# Autodesk Inventor assembly: Frame
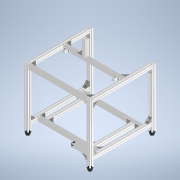
[picture p0: Inventor's stored thumbnail of the model, 180x180]
Saved by Autodesk Inventor 2020.2 (Build 242310000, 310)
## iProperties
Created: 2020-07-30
Part Number: Frame
Document SubType Name: Assembly
Designer: JK
Author: JK
## Documents named in this file (10)
- C:\Users\JK\Documents\Inventor\Anet Upgrade\Frame.iam
- C:\Users\JK\Documents\Inventor\Anet Upgrade\30x30x500.ipt
- C:\Users\JK\Documents\Inventor\Anet Upgrade\Cornerassembly.iam
- C:\Users\JK\Documents\Inventor\Anet Upgrade\SK8.iam
- C:\Users\JK\Documents\Inventor\Anet Upgrade\30x30x125.ipt
- C:\Users\JK\Documents\Inventor\Anet Upgrade\30x30x340.ipt
- C:\Users\JK\Documents\Inventor\Anet Upgrade\3030_endCap.ipt
- C:\Users\JK\Documents\Inventor\Anet Upgrade\Footassembly.iam
- C:\Users\JK\Documents\Inventor\Anet Upgrade\M5x12BoltFlatHead.ipt
- C:\Users\JK\Documents\Inventor\Anet Upgrade\T_Slot_Nut_Dropin_3030m5ipt.ipt
## Components (53 placed, 9 different names)
1. 30x30x500:9 — Flush:17, Mate:14, Flush:19, Flush:24, Mate:38, Mate:42
2. 30x30x500:10 — Flush:16, Flush:17, Mate:13, Flush:18, Mate:36, Mate:40, Flush:57
3. 30x30x500:3 — Mate:12, Flush:16, Mate:49, Flush:51, Mate:50, Flush:52, Mate:55, Mate:58, Flush:56, Flush:64, Mate:88
4. 30x30x500:4 — Mate:12, Mate:51, Mate:53
5. Cornerassembly:1 [sub-assembly]
6. Cornerassembly:2 [sub-assembly]
7. Cornerassembly:3 [sub-assembly]
8. Cornerassembly:4 [sub-assembly]
9. 30x30x500:1 — Mate:13, Flush:18, Mate:17, Flush:25, Mate:34, Mate:41, Flush:45, Mate:66, Mate:67, Flush:62, Mate:73, Angle:1, Mate:83, Flush:78
10. 30x30x500:2 — Mate:14, Flush:19, Flush:27, Mate:28, Flush:39, Flush:46, Mate:60, Mate:61, Flush:58, Flush:59, Mate:75, Angle:4, Flush:77, Mate:85, Mate:88
11. 30x30x500:5 — Flush:24, Mate:18, Mate:30, Mate:39, Flush:44, Mate:82, Flush:80
12. 30x30x500:6 — Flush:79, Flush:81, Flush:82, Mate:87, Mate:89, Flush:85, Mate:90, Mate:95
13. 30x30x500:11 — Mate:17, Flush:25, Mate:19, Mate:27, Flush:41, Flush:42, Mate:64, Flush:61, Flush:81, Flush:82, Mate:89, Mate:94, Flush:87, Mate:101
14. 30x30x500:12 — Mate:18, Flush:27, Flush:40, Flush:50, Mate:63, Flush:77, Mate:85, Flush:80, Flush:83, Mate:91, Mate:93, Angle:5, Mate:102
15. 30x30x500:7 — Mate:19, Mate:20, Flush:31, Mate:26, Flush:38, Mate:45, Flush:48, Flush:83, Flush:84, Mate:86, Flush:86, Mate:92, Flush:91
16. SK8:1 [sub-assembly] — Mate:20, Flush:31, Mate:79, Mate:80, Flush:76, Mate:84, Mate:96, Angle:5, Angle:6
17. SK8:2 [sub-assembly] — Mate:60, Mate:78, Mate:81, Flush:76, Mate:96, Flush:87, Angle:7, Angle:8
18. Cornerassembly:5 [sub-assembly] — Flush:86, Mate:92, Mate:93
19. Cornerassembly:6 [sub-assembly] — Mate:26, Mate:27, Flush:38
20. Cornerassembly:7 [sub-assembly] — Mate:28, Flush:39, Mate:102
21. Cornerassembly:8 [sub-assembly] — Mate:30, Flush:40, Mate:91
22. Cornerassembly:9 [sub-assembly] — Flush:41, Mate:94, Mate:95
23. Cornerassembly:10 [sub-assembly] — Mate:34, Flush:42, Mate:101
24. Cornerassembly:11 [sub-assembly] — Mate:36, Flush:85, Mate:90
25. Cornerassembly:13 [sub-assembly] — Mate:40, Mate:41, Flush:45
26. Cornerassembly:14 [sub-assembly] — Mate:38, Mate:39, Flush:44
27. Cornerassembly:15 [sub-assembly] — Mate:42, Flush:46
28. 30x30x125:1 — Mate:46, Flush:50, Flush:84, Mate:86
29. Cornerassembly:16 [sub-assembly] — Mate:45, Mate:46, Flush:48
30. 30x30x340:1 — Mate:49, Flush:51, Flush:54, Mate:54, Flush:55, Mate:56, Mate:59
31. 30x30x340:2 — Mate:50, Flush:52, Mate:52, Flush:53, Mate:57, Mate:59, Flush:57
32. Cornerassembly:17 [sub-assembly] — Flush:54, Mate:53, Mate:54
33. Cornerassembly:18 [sub-assembly] — Mate:57, Mate:58, Flush:56
34. Cornerassembly:19 [sub-assembly] — Mate:55, Flush:55, Mate:56
35. Cornerassembly:20 [sub-assembly] — Mate:51, Mate:52, Flush:53
36. 30x30x500:8 — Mate:61, Flush:58, Flush:59, Mate:62, Flush:60, Flush:78, Flush:79
37. Cornerassembly:21 [sub-assembly] — Mate:62, Flush:60, Mate:63
38. Cornerassembly:22 [sub-assembly] — Mate:64, Flush:61
39. Cornerassembly:23 [sub-assembly] — Mate:66, Mate:68, Flush:63, Flush:64
40. 30x30x125:2 — Mate:67, Flush:62, Mate:68, Flush:63, Mate:69, Flush:65, Flush:66
41. 3030_endCap:1 — Mate:69, Flush:65, Flush:66
42. Footassembly:1 [sub-assembly] — Mate:73, Angle:1, Flush:69, Flush:70, Flush:75, Mate:83
43. Footassembly:2 [sub-assembly] — Mate:75, Flush:69, Angle:4
44. Footassembly:3 [sub-assembly] — Flush:75, Mate:82
45. Footassembly:4 [sub-assembly] — Flush:70, Mate:87
46. M5x12BoltFlatHead:1 — Mate:78, Flush:72, Flush:73, Mate:100
47. M5x12BoltFlatHead:2 — Mate:79, Flush:74, Mate:98
48. M5x12BoltFlatHead:3 — Mate:80, Flush:73, Flush:74, Mate:84, Mate:97
49. M5x12BoltFlatHead:4 — Mate:81, Flush:72, Mate:99
50. T_Slot_Nut_Dropin_3030m5ipt:1 — Mate:97, Flush:90, Angle:6
51. T_Slot_Nut_Dropin_3030m5ipt:2 — Mate:98, Flush:89, Flush:90
52. T_Slot_Nut_Dropin_3030m5ipt:3 — Mate:99, Flush:88, Flush:89, Angle:7, Flush:91
53. T_Slot_Nut_Dropin_3030m5ipt:4 — Mate:100, Flush:88, Angle:8
## Relationships (147: Mate 78, Flush 63, Angle 6)
- [Mate]: 30x30x500:9 ↔ 30x30x500:3
- [Flush]: 30x30x500:9 ↔ 30x30x500:3
- [Mate]: 30x30x500:9 ↔ 30x30x500:4
- [Flush]: 30x30x500:9 ↔ 30x30x500:4
- [Mate]: 30x30x500:10 ↔ 30x30x500:3
- [Flush]: 30x30x500:10 ↔ 30x30x500:4
- [Mate]: 30x30x500:9 ↔ Cornerassembly:1
- [Mate]: 30x30x500:4 ↔ Cornerassembly:1
- [Flush] (0.5 mm): 30x30x500:9 ↔ Cornerassembly:1
- [Mate]: 30x30x500:3 ↔ Cornerassembly:3
- [Flush] (0.5 mm): 30x30x500:9 ↔ Cornerassembly:3
- [Mate]: 30x30x500:9 ↔ Cornerassembly:3
- [Mate]: 30x30x500:3 ↔ Cornerassembly:2
- [Mate]: 30x30x500:10 ↔ Cornerassembly:2
- [Flush] (0.5 mm): 30x30x500:10 ↔ Cornerassembly:2
- [Mate]: 30x30x500:10 ↔ Cornerassembly:4
- [Mate]: 30x30x500:4 ↔ Cornerassembly:4
- [Flush] (0.5 mm): 30x30x500:4 ↔ Cornerassembly:4
- Mate:12 (-400 mm): 30x30x500:3 ↔ 30x30x500:4
- Flush:16 (-50 mm): 30x30x500:10 ↔ 30x30x500:3
- Flush:17: 30x30x500:9 ↔ 30x30x500:10
- Mate:13: 30x30x500:10 ↔ 30x30x500:1
- Mate:14: 30x30x500:9 ↔ 30x30x500:2
- Flush:18: 30x30x500:10 ↔ 30x30x500:1
- Flush:19: 30x30x500:9 ↔ 30x30x500:2
- Flush:24: 30x30x500:9 ↔ 30x30x500:5
- Mate:17: 30x30x500:1 ↔ 30x30x500:11
- Flush:25: 30x30x500:1 ↔ 30x30x500:11
- Mate:18: 30x30x500:5 ↔ 30x30x500:12
- Flush:27: 30x30x500:2 ↔ 30x30x500:12
- Mate:19: 30x30x500:11 ↔ 30x30x500:7
- Mate:20: 30x30x500:7 ↔ SK8:1
- Flush:31 (8 mm): 30x30x500:7 ↔ SK8:1
- Mate:26: 30x30x500:7 ↔ Cornerassembly:6
- Mate:27: 30x30x500:11 ↔ Cornerassembly:6
- Flush:38 (0.5 mm): 30x30x500:7 ↔ Cornerassembly:6
- Mate:28: 30x30x500:2 ↔ Cornerassembly:7
- Flush:39 (0.5 mm): 30x30x500:2 ↔ Cornerassembly:7
- Mate:30: 30x30x500:5 ↔ Cornerassembly:8
- Flush:40 (0.5 mm): 30x30x500:12 ↔ Cornerassembly:8
- Flush:41 (0.5 mm): 30x30x500:11 ↔ Cornerassembly:9
- Mate:34: 30x30x500:1 ↔ Cornerassembly:10
- Flush:42 (0.5 mm): 30x30x500:11 ↔ Cornerassembly:10
- Mate:36: 30x30x500:10 ↔ Cornerassembly:11
- Mate:38: 30x30x500:9 ↔ Cornerassembly:14
- Mate:39: 30x30x500:5 ↔ Cornerassembly:14
- Flush:44 (0.5 mm): 30x30x500:5 ↔ Cornerassembly:14
- Mate:40: 30x30x500:10 ↔ Cornerassembly:13
- Mate:41: 30x30x500:1 ↔ Cornerassembly:13
- Flush:45 (0.5 mm): 30x30x500:1 ↔ Cornerassembly:13
- Mate:42: 30x30x500:9 ↔ Cornerassembly:15
- Flush:46 (0.5 mm): 30x30x500:2 ↔ Cornerassembly:15
- Mate:45: 30x30x500:7 ↔ Cornerassembly:16
- Mate:46: 30x30x125:1 ↔ Cornerassembly:16
- Flush:48 (0.5 mm): 30x30x500:7 ↔ Cornerassembly:16
- Flush:50 (190 mm): 30x30x500:12 ↔ 30x30x125:1
- Mate:49: 30x30x500:3 ↔ 30x30x340:1
- Flush:51: 30x30x500:3 ↔ 30x30x340:1
- Mate:50: 30x30x500:3 ↔ 30x30x340:2
- Flush:52: 30x30x500:3 ↔ 30x30x340:2
- Mate:51: 30x30x500:4 ↔ Cornerassembly:20
- Mate:52: 30x30x340:2 ↔ Cornerassembly:20
- Flush:53: 30x30x340:2 ↔ Cornerassembly:20
- Flush:54 (0.5 mm): 30x30x340:1 ↔ Cornerassembly:17
- Mate:53: 30x30x500:4 ↔ Cornerassembly:17
- Mate:54: 30x30x340:1 ↔ Cornerassembly:17
- Mate:55: 30x30x500:3 ↔ Cornerassembly:19
- Flush:55 (0.5 mm): 30x30x340:1 ↔ Cornerassembly:19
- Mate:56: 30x30x340:1 ↔ Cornerassembly:19
- Mate:57: 30x30x340:2 ↔ Cornerassembly:18
- Mate:58: 30x30x500:3 ↔ Cornerassembly:18
- Flush:56 (0.5 mm): 30x30x500:3 ↔ Cornerassembly:18
- Mate:59 (362 mm): 30x30x340:1 ↔ 30x30x340:2
- Flush:57 (69 mm): 30x30x500:10 ↔ 30x30x340:2
- Mate:60 (-280 mm): 30x30x500:2 ↔ SK8:2
- Mate:61: 30x30x500:2 ↔ 30x30x500:8
- Flush:58: 30x30x500:2 ↔ 30x30x500:8
- Flush:59: 30x30x500:2 ↔ 30x30x500:8
- Mate:62: 30x30x500:8 ↔ Cornerassembly:21
- Flush:60 (0.5 mm): 30x30x500:8 ↔ Cornerassembly:21
- Mate:63: 30x30x500:12 ↔ Cornerassembly:21
- Mate:64: 30x30x500:11 ↔ Cornerassembly:22
- Flush:61 (0.5 mm): 30x30x500:11 ↔ Cornerassembly:22
- Mate:66: 30x30x500:1 ↔ Cornerassembly:23
- Mate:67: 30x30x500:1 ↔ 30x30x125:2
- Flush:62: 30x30x500:1 ↔ 30x30x125:2
- Mate:68: Cornerassembly:23 ↔ 30x30x125:2
- Flush:63 (0.5 mm): Cornerassembly:23 ↔ 30x30x125:2
- Flush:64: 30x30x500:3 ↔ Cornerassembly:23
- Mate:69: 30x30x125:2 ↔ 3030_endCap:1
- Flush:65: 30x30x125:2 ↔ 3030_endCap:1
- Flush:66: 30x30x125:2 ↔ 3030_endCap:1
- Mate:73: 30x30x500:1 ↔ Footassembly:1
- Angle:1 (0 deg): 30x30x500:1 ↔ Footassembly:1
- Mate:75: 30x30x500:2 ↔ Footassembly:2
- Flush:69: Footassembly:1 ↔ Footassembly:2
- Flush:70: Footassembly:1 ↔ Footassembly:4
- Angle:4 (0 deg): 30x30x500:2 ↔ Footassembly:2
- Mate:78: SK8:2 ↔ M5x12BoltFlatHead:1
- Mate:79: SK8:1 ↔ M5x12BoltFlatHead:2
- Mate:80: SK8:1 ↔ M5x12BoltFlatHead:3
- Mate:81: SK8:2 ↔ M5x12BoltFlatHead:4
- Flush:72: M5x12BoltFlatHead:1 ↔ M5x12BoltFlatHead:4
- Flush:73: M5x12BoltFlatHead:1 ↔ M5x12BoltFlatHead:3
- Flush:74: M5x12BoltFlatHead:2 ↔ M5x12BoltFlatHead:3
- Flush:75: Footassembly:1 ↔ Footassembly:3
- Mate:82: 30x30x500:5 ↔ Footassembly:3
- Mate:83: 30x30x500:1 ↔ Footassembly:1
- Flush:76: SK8:1 ↔ SK8:2
- Mate:84: SK8:1 ↔ M5x12BoltFlatHead:3
- Flush:77: 30x30x500:2 ↔ 30x30x500:12
- Mate:85: 30x30x500:2 ↔ 30x30x500:12
- Flush:78: 30x30x500:1 ↔ 30x30x500:8
- Flush:79: 30x30x500:6 ↔ 30x30x500:8
- Flush:80: 30x30x500:5 ↔ 30x30x500:12
- Flush:81: 30x30x500:6 ↔ 30x30x500:11
- Flush:82: 30x30x500:6 ↔ 30x30x500:11
- Flush:83: 30x30x500:12 ↔ 30x30x500:7
- Flush:84: 30x30x500:7 ↔ 30x30x125:1
- Mate:86: 30x30x500:7 ↔ 30x30x125:1
- Mate:87: 30x30x500:6 ↔ Footassembly:4
- Mate:88 (47 mm): 30x30x500:3 ↔ 30x30x500:2
- Mate:89: 30x30x500:6 ↔ 30x30x500:11
- Flush:85 (0.5 mm): 30x30x500:6 ↔ Cornerassembly:11
- Mate:90: 30x30x500:6 ↔ Cornerassembly:11
- Mate:91: 30x30x500:12 ↔ Cornerassembly:8
- Flush:86 (0.5 mm): 30x30x500:7 ↔ Cornerassembly:5
- Mate:92: 30x30x500:7 ↔ Cornerassembly:5
- Mate:93: 30x30x500:12 ↔ Cornerassembly:5
- Mate:94: 30x30x500:11 ↔ Cornerassembly:9
- Mate:95: 30x30x500:6 ↔ Cornerassembly:9
- Mate:96 (423.5 mm): SK8:1 ↔ SK8:2
- Flush:87 (47.5 mm): 30x30x500:11 ↔ SK8:2
- Mate:97: M5x12BoltFlatHead:3 ↔ T_Slot_Nut_Dropin_3030m5ipt:1
- Mate:98: M5x12BoltFlatHead:2 ↔ T_Slot_Nut_Dropin_3030m5ipt:2
- Mate:99: M5x12BoltFlatHead:4 ↔ T_Slot_Nut_Dropin_3030m5ipt:3
- Mate:100: M5x12BoltFlatHead:1 ↔ T_Slot_Nut_Dropin_3030m5ipt:4
- Flush:88: T_Slot_Nut_Dropin_3030m5ipt:3 ↔ T_Slot_Nut_Dropin_3030m5ipt:4
- Flush:89: T_Slot_Nut_Dropin_3030m5ipt:2 ↔ T_Slot_Nut_Dropin_3030m5ipt:3
- Flush:90: T_Slot_Nut_Dropin_3030m5ipt:1 ↔ T_Slot_Nut_Dropin_3030m5ipt:2
- Angle:5 (0 deg): 30x30x500:12 ↔ SK8:1
- Angle:6 (0 deg): SK8:1 ↔ T_Slot_Nut_Dropin_3030m5ipt:1
- Angle:7 (0 deg): SK8:2 ↔ T_Slot_Nut_Dropin_3030m5ipt:3
- Angle:8 (0 deg): SK8:2 ↔ T_Slot_Nut_Dropin_3030m5ipt:4
- Flush:91: 30x30x500:7 ↔ T_Slot_Nut_Dropin_3030m5ipt:3
- Mate:101: 30x30x500:11 ↔ Cornerassembly:10
- Mate:102: 30x30x500:12 ↔ Cornerassembly:7
